# Autodesk Inventor assembly: 3_left_leg_true_final
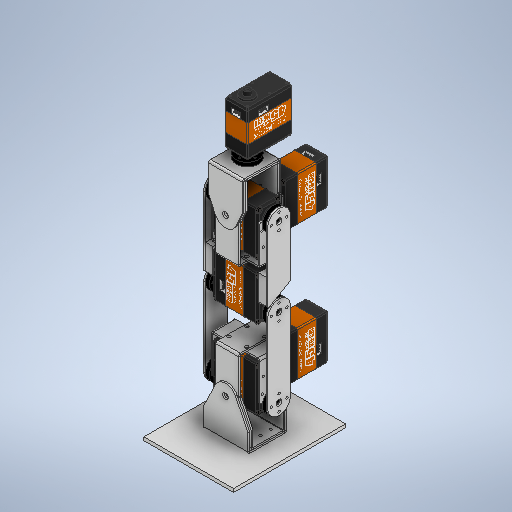
[picture p0: Inventor's stored thumbnail of the model, 512x512]
Saved by Autodesk Inventor 2025.2 (Build 292293000, 293)
## iProperties
Created: 2025-08-03
Part Number: 3_left_leg_true_final
Document SubType Name: Assembly
Designer: User
Author: User
## Documents named in this file (19)
- C:\Users\User\Documents\The Maverick's Files\College 3-3\로보인 프로젝트\RHp_Humanoid_ver1\Assembly\3_left_leg_true_final.iam
- C:\Users\User\Documents\The Maverick's Files\College 3-3\로보인 프로젝트\RHp_Humanoid_ver1\Part\HTD-45H, Horn\HTD-45H\HTD-45H.iam
- C:\Users\User\Documents\The Maverick's Files\College 3-3\로보인 프로젝트\RHp_Humanoid_ver1\Part\HTD-45H, Horn\Horn\Top Horn.ipt
- C:\Users\User\Documents\The Maverick's Files\College 3-3\로보인 프로젝트\RHp_Humanoid_ver1\Part\HTD-45H, Horn\Horn\Bottom Horn.ipt
- C:\Users\User\Documents\The Maverick's Files\College 3-3\로보인 프로젝트\RHp_Humanoid_ver1\Part\Frame\Leg\Left Leg\axis_1_top_frame.ipt
- C:\Users\User\Documents\The Maverick's Files\College 3-3\로보인 프로젝트\RHp_Humanoid_ver1\Part\Frame\Leg\Left Leg\axis_3_bottom_frame.ipt
- C:\Users\User\Documents\The Maverick's Files\College 3-3\로보인 프로젝트\RHp_Humanoid_ver1\Part\Frame\Leg\Left Leg\axis_2_bottom_frame.ipt
- C:\Users\User\Documents\The Maverick's Files\College 3-3\로보인 프로젝트\RHp_Humanoid_ver1\Part\Frame\Leg\Left Leg\axis_1_supplement_frame.ipt
- C:\Users\User\Documents\The Maverick's Files\College 3-3\로보인 프로젝트\RHp_Humanoid_ver1\Part\Frame\Leg\Left Leg\axis_2_4_connector_frame_powered.ipt
- C:\Users\User\Documents\The Maverick's Files\College 3-3\로보인 프로젝트\RHp_Humanoid_ver1\Part\Frame\Leg\Left Leg\axis_2_4_connector_frame_non_powered.ipt
- C:\Users\User\Documents\The Maverick's Files\College 3-3\로보인 프로젝트\RHp_Humanoid_ver1\Part\Frame\Leg\3D_printed_part_powered.ipt
- C:\Users\User\Documents\The Maverick's Files\College 3-3\로보인 프로젝트\RHp_Humanoid_ver1\Part\Frame\Leg\3D_printed_part_non_powered.ipt
- C:\Users\User\Documents\The Maverick's Files\College 3-3\로보인 프로젝트\RHp_Humanoid_ver1\Part\Frame\Leg\Left Leg\axis_4_5_connector_frame_powered.ipt
- C:\Users\User\Documents\The Maverick's Files\College 3-3\로보인 프로젝트\RHp_Humanoid_ver1\Part\Frame\Leg\Left Leg\axis_4_5_connector_frame_non_powered.ipt
- C:\Users\User\Documents\The Maverick's Files\College 3-3\로보인 프로젝트\RHp_Humanoid_ver1\Part\Frame\Leg\Left Leg\axis_5_top_frame.ipt
- C:\Users\User\Documents\The Maverick's Files\College 3-3\로보인 프로젝트\RHp_Humanoid_ver1\Part\Frame\Leg\Left Leg\axis_6_top_frame.ipt
- C:\Users\User\Documents\The Maverick's Files\College 3-3\로보인 프로젝트\RHp_Humanoid_ver1\Part\Frame\Leg\Left Leg\axis_6_bottom_frame(top).ipt
- C:\Users\User\Documents\The Maverick's Files\College 3-3\로보인 프로젝트\RHp_Humanoid_ver1\Part\Frame\Leg\Left Leg\axis_6_bottom_frame(bottom).ipt
- C:\Users\User\Documents\The Maverick's Files\College 3-3\로보인 프로젝트\RHp_Humanoid_ver1\Part\Frame\Leg\Left Leg\axis_6_supplement_frame.ipt
## Components (30 placed, 18 different names)
1. axis_1_supplement_frame:1 — Rigid:5
2. axis_1_top_frame:1 — Rigid:1, Rigid:2, Rigid:5
3. Top Horn:1 — Rotational:1, Rigid:1
4. HTD-45H:1 [sub-assembly] — Rotational:1
5. axis_2_bottom_frame:1 — Rigid:4, Rigid:6
6. axis_2_4_connector_frame_powered:1 — Rigid:7, Rigid:23
7. axis_2_4_connector_frame_non_powered:1 — Rigid:8, Rigid:24
8. Top Horn:2 — Rotational:2, Rigid:2
9. HTD-45H:3 [sub-assembly] — Rotational:3, Rigid:4
10. Bottom Horn:3 — Rigid:8
11. Top Horn:3 — Rotational:3, Rigid:7
12. axis_3_bottom_frame:1 — Rigid:3, Rigid:6
13. HTD-45H:2 [sub-assembly] — Rotational:2, Rigid:3
14. Bottom Horn:4 — Rotational:6, Rigid:13
15. Top Horn:4 — Rotational:5, Rigid:12
16. HTD-45H:4 [sub-assembly] — Rotational:5, Rotational:6, Rigid:11, Rigid:21
17. 3D_printed_part_powered:1 — Rigid:11, Rigid:23
18. 3D_printed_part_non_powered:1 — Rigid:21, Rigid:24
19. axis_4_5_connector_frame_powered:1 — Rigid:12, Rigid:15
20. axis_4_5_connector_frame_non_powered:1 — Rigid:13, Rigid:22
21. HTD-45H:5 [sub-assembly] — Rotational:7, Rotational:8, Rigid:14
22. Bottom Horn:5 — Rotational:8, Rigid:22
23. Top Horn:5 — Rotational:7, Rigid:15
24. axis_5_top_frame:1 — Rigid:14, Rigid:17
25. Top Horn:6 — Rotational:9, Rigid:19
26. HTD-45H:6 [sub-assembly] — Rigid:16, Rotational:9
27. axis_6_top_frame:1 — Rigid:16, Rigid:17
28. axis_6_bottom_frame(top):1 — Rigid:18, Rigid:19, Rigid:20
29. axis_6_bottom_frame(bottom):1 — Rigid:20
30. axis_6_supplement_frame:1 — Rigid:18
## Relationships (30: WeldJoint 22, RevoluteJoint 8)
- Rotational:1 [RevoluteJoint]: Top Horn:1 ↔ HTD-45H:1
- Rigid:1 [WeldJoint]: axis_1_top_frame:1 ↔ Top Horn:1
- Rotational:2 [RevoluteJoint]: Top Horn:2 ↔ HTD-45H:2
- Rigid:2 [WeldJoint]: axis_1_top_frame:1 ↔ Top Horn:2
- Rigid:3 [WeldJoint]: axis_3_bottom_frame:1 ↔ HTD-45H:2
- Rotational:3 [RevoluteJoint]: HTD-45H:3 ↔ Top Horn:3
- Rigid:4 [WeldJoint]: axis_2_bottom_frame:1 ↔ HTD-45H:3
- Rigid:5 [WeldJoint]: axis_1_supplement_frame:1 ↔ axis_1_top_frame:1
- Rigid:6 [WeldJoint]: axis_2_bottom_frame:1 ↔ axis_3_bottom_frame:1
- Rigid:7 [WeldJoint]: axis_2_4_connector_frame_powered:1 ↔ Top Horn:3
- Rigid:8 [WeldJoint]: axis_2_4_connector_frame_non_powered:1 ↔ Bottom Horn:3
- Rotational:5 [RevoluteJoint]: Top Horn:4 ↔ HTD-45H:4
- Rotational:6 [RevoluteJoint]: Bottom Horn:4 ↔ HTD-45H:4
- Rigid:11 [WeldJoint]: HTD-45H:4 ↔ 3D_printed_part_powered:1
- Rigid:12 [WeldJoint]: Top Horn:4 ↔ axis_4_5_connector_frame_powered:1
- Rigid:13 [WeldJoint]: Bottom Horn:4 ↔ axis_4_5_connector_frame_non_powered:1
- Rotational:7 [RevoluteJoint]: HTD-45H:5 ↔ Top Horn:5
- Rotational:8 [RevoluteJoint]: HTD-45H:5 ↔ Bottom Horn:5
- Rigid:14 [WeldJoint]: HTD-45H:5 ↔ axis_5_top_frame:1
- Rigid:15 [WeldJoint]: axis_4_5_connector_frame_powered:1 ↔ Top Horn:5
- Rigid:16 [WeldJoint]: HTD-45H:6 ↔ axis_6_top_frame:1
- Rotational:9 [RevoluteJoint]: Top Horn:6 ↔ HTD-45H:6
- Rigid:17 [WeldJoint]: axis_5_top_frame:1 ↔ axis_6_top_frame:1
- Rigid:18 [WeldJoint]: axis_6_bottom_frame(top):1 ↔ axis_6_supplement_frame:1
- Rigid:19 [WeldJoint]: Top Horn:6 ↔ axis_6_bottom_frame(top):1
- Rigid:20 [WeldJoint]: axis_6_bottom_frame(top):1 ↔ axis_6_bottom_frame(bottom):1
- Rigid:21 [WeldJoint]: HTD-45H:4 ↔ 3D_printed_part_non_powered:1
- Rigid:22 [WeldJoint]: axis_4_5_connector_frame_non_powered:1 ↔ Bottom Horn:5
- Rigid:23 [WeldJoint]: axis_2_4_connector_frame_powered:1 ↔ 3D_printed_part_powered:1
- Rigid:24 [WeldJoint]: axis_2_4_connector_frame_non_powered:1 ↔ 3D_printed_part_non_powered:1
